# Autodesk Inventor assembly: Joint Assembly
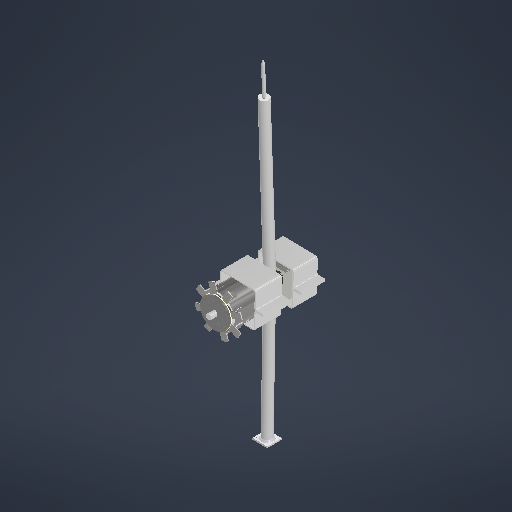
[picture p0: Inventor's stored thumbnail of the model, 512x512]
Saved by Autodesk Inventor 2026.3 (Build 303398000, 398)
## iProperties
Created: 2026-07-22
Part Number: Joint Assembly
Document SubType Name: Assembly
Designer: matot
Author: matot
## Documents named in this file (16)
- C:\Users\matot\OneDrive - Stellenbosch University\2026\MechatronicsProject478\Building the joint\Joint Assembly\Joint Assembly.iam
- C:\Users\matot\OneDrive - Stellenbosch University\2026\MechatronicsProject478\Building the joint\Joint Assembly\Final joint shaft.ipt
- C:\Users\matot\OneDrive - Stellenbosch University\2026\MechatronicsProject478\Building the joint\Joint Assembly\2058786.iam
- C:\Users\matot\OneDrive - Stellenbosch University\2026\MechatronicsProject478\Building the joint\Joint Assembly\8236967.ipt
- C:\Users\matot\OneDrive - Stellenbosch University\2026\MechatronicsProject478\Building the joint\Joint Assembly\Optical Encoder.ipt
- C:\Users\matot\OneDrive - Stellenbosch University\2026\MechatronicsProject478\Building the joint\Joint Assembly\Electromagnet final.iam
- C:\Users\matot\OneDrive - Stellenbosch University\2026\MechatronicsProject478\Building the joint\Joint Assembly\Pressure platform.ipt
- C:\Users\matot\OneDrive - Stellenbosch University\2026\MechatronicsProject478\Building the joint\Joint Assembly\Friction Plate.ipt
- C:\Users\matot\OneDrive - Stellenbosch University\2026\MechatronicsProject478\Building the joint\Joint Assembly\Brake disc.ipt
- C:\Users\matot\OneDrive - Stellenbosch University\2026\MechatronicsProject478\Building the joint\Joint Assembly\Bearing housing top.ipt
- C:\Users\matot\OneDrive - Stellenbosch University\2026\MechatronicsProject478\Building the joint\Joint Assembly\Bearing housing bottom.ipt
- C:\Users\matot\OneDrive - Stellenbosch University\2026\MechatronicsProject478\Building the joint\Joint Assembly\Joint Housing Bottom_final.iam
- C:\Users\matot\OneDrive - Stellenbosch University\2026\MechatronicsProject478\Building the joint\Joint Assembly\Complete front top housing.iam
- C:\Users\matot\OneDrive - Stellenbosch University\2026\MechatronicsProject478\Building the joint\Joint Assembly\Complete back top housing.iam
- C:\Users\matot\OneDrive - Stellenbosch University\2026\MechatronicsProject478\Building the joint\Joint Assembly\Base link.iam
- C:\Users\matot\OneDrive - Stellenbosch University\2026\MechatronicsProject478\Building the joint\Joint Assembly\Output Link.iam
## Components (26 placed, 15 different names)
1. Final joint shaft:1 — Insert:1, Insert:2, Mate:1, Insert:5, Flush:9, Insert:15, Insert:16, Tangent:3, Mate:17, Tangent:4
2. 2058786:1 [sub-assembly] — Insert:2, Insert:4, Insert:17, Insert:20
3. 2058786:2 [sub-assembly] — Insert:1, Insert:3, Insert:18, Insert:19
4. 8236967:1 — Insert:4, Insert:6
5. 8236967:2 — Insert:3
6. Optical Encoder:1 — Mate:1, Insert:5
7. Electromagnet final:3 [sub-assembly] — Insert:6, Mate:2, Insert:7, Flush:1, Mate:3, Insert:8, Flush:2, Mate:4, Insert:9, Flush:3, Mate:5, Insert:10, Flush:4, Mate:6, Insert:11, Flush:5, Mate:7, Insert:12, Flush:6, Mate:8, Insert:13, Flush:7, Mate:9, Insert:14, Flush:8, Tangent:1, Tangent:2, Flush:10
8. Pressure platform:2 — Mate:3, Insert:8, Flush:2
9. Pressure platform:3 — Mate:4, Insert:9, Flush:3
10. Pressure platform:4 — Mate:5, Insert:10, Flush:4
11. Pressure platform:5 — Mate:2, Insert:7, Flush:1
12. Pressure platform:6 — Mate:6, Insert:11, Flush:5
13. Pressure platform:7 — Mate:9, Insert:14, Flush:8
14. Pressure platform:8 — Mate:8, Insert:13, Flush:7
15. Pressure platform:9 — Mate:7, Insert:12, Flush:6
16. Friction Plate:1 — Flush:9, Insert:15, Mate:10
17. Brake disc:1 — Mate:10, Insert:16
18. Bearing housing top:1 — Insert:17, Mate:14
19. Bearing housing top:2 — Insert:18, Mate:13
20. Bearing housing bottom:1 — Insert:20, Mate:14, Mate:15
21. Bearing housing bottom:2 — Insert:19, Mate:13, Mate:16
22. Joint Housing Bottom_final:2 [sub-assembly] — Tangent:1, Tangent:2, Flush:10, Mate:11, Flush:11, Flush:12, Flush:13, Mate:12, Flush:14, Mate:15, Mate:16, Insert:21, Insert:22
23. Complete front top housing:1 [sub-assembly] — Mate:11, Flush:11, Flush:12
24. Complete back top housing:1 [sub-assembly] — Flush:13, Mate:12, Flush:14
25. Base link:1 [sub-assembly] — Insert:21, Insert:22
26. Output Link:1 [sub-assembly] — Tangent:3, Mate:17, Tangent:4
## Relationships (57: Insert 22, Mate 17, Flush 14, Tangent 4)
- Insert:1: Final joint shaft:1 ↔ 2058786:2
- Insert:2: Final joint shaft:1 ↔ 2058786:1
- Insert:3: 2058786:2 ↔ 8236967:2
- Insert:4: 2058786:1 ↔ 8236967:1
- Mate:1: Final joint shaft:1 ↔ Optical Encoder:1
- Insert:5: Final joint shaft:1 ↔ Optical Encoder:1
- Insert:6 (5 mm): 8236967:1 ↔ Electromagnet final:3
- Mate:2: Electromagnet final:3 ↔ Pressure platform:5
- Insert:7: Electromagnet final:3 ↔ Pressure platform:5
- Flush:1: Electromagnet final:3 ↔ Pressure platform:5
- Mate:3: Electromagnet final:3 ↔ Pressure platform:2
- Insert:8: Electromagnet final:3 ↔ Pressure platform:2
- Flush:2: Electromagnet final:3 ↔ Pressure platform:2
- Mate:4: Electromagnet final:3 ↔ Pressure platform:3
- Insert:9: Electromagnet final:3 ↔ Pressure platform:3
- Flush:3: Electromagnet final:3 ↔ Pressure platform:3
- Mate:5: Electromagnet final:3 ↔ Pressure platform:4
- Insert:10: Electromagnet final:3 ↔ Pressure platform:4
- Flush:4: Electromagnet final:3 ↔ Pressure platform:4
- Mate:6: Electromagnet final:3 ↔ Pressure platform:6
- Insert:11: Electromagnet final:3 ↔ Pressure platform:6
- Flush:5: Electromagnet final:3 ↔ Pressure platform:6
- Mate:7: Electromagnet final:3 ↔ Pressure platform:9
- Insert:12: Electromagnet final:3 ↔ Pressure platform:9
- Flush:6: Electromagnet final:3 ↔ Pressure platform:9
- Mate:8: Electromagnet final:3 ↔ Pressure platform:8
- Insert:13: Electromagnet final:3 ↔ Pressure platform:8
- Flush:7: Electromagnet final:3 ↔ Pressure platform:8
- Mate:9: Electromagnet final:3 ↔ Pressure platform:7
- Insert:14: Electromagnet final:3 ↔ Pressure platform:7
- Flush:8: Electromagnet final:3 ↔ Pressure platform:7
- Flush:9: Final joint shaft:1 ↔ Friction Plate:1
- Insert:15: Final joint shaft:1 ↔ Friction Plate:1
- Mate:10: Friction Plate:1 ↔ Brake disc:1
- Insert:16: Final joint shaft:1 ↔ Brake disc:1
- Insert:17: 2058786:1 ↔ Bearing housing top:1
- Insert:18: 2058786:2 ↔ Bearing housing top:2
- Insert:19: 2058786:2 ↔ Bearing housing bottom:2
- Insert:20: 2058786:1 ↔ Bearing housing bottom:1
- Tangent:1: Electromagnet final:3 ↔ Joint Housing Bottom_final:2
- Tangent:2: Electromagnet final:3 ↔ Joint Housing Bottom_final:2
- Flush:10 (-65 mm): Electromagnet final:3 ↔ Joint Housing Bottom_final:2
- Mate:11: Joint Housing Bottom_final:2 ↔ Complete front top housing:1
- Flush:11: Joint Housing Bottom_final:2 ↔ Complete front top housing:1
- Flush:12: Joint Housing Bottom_final:2 ↔ Complete front top housing:1
- Flush:13: Joint Housing Bottom_final:2 ↔ Complete back top housing:1
- Mate:12: Joint Housing Bottom_final:2 ↔ Complete back top housing:1
- Flush:14: Joint Housing Bottom_final:2 ↔ Complete back top housing:1
- Mate:13: Bearing housing top:2 ↔ Bearing housing bottom:2
- Mate:14: Bearing housing top:1 ↔ Bearing housing bottom:1
- Mate:15: Bearing housing bottom:1 ↔ Joint Housing Bottom_final:2
- Mate:16: Bearing housing bottom:2 ↔ Joint Housing Bottom_final:2
- Insert:21: Joint Housing Bottom_final:2 ↔ Base link:1
- Insert:22: Joint Housing Bottom_final:2 ↔ Base link:1
- Tangent:3: Final joint shaft:1 ↔ Output Link:1
- Mate:17: Final joint shaft:1 ↔ Output Link:1
- Tangent:4: Final joint shaft:1 ↔ Output Link:1
